# Autodesk Inventor assembly: UQ204-topHolder-sample
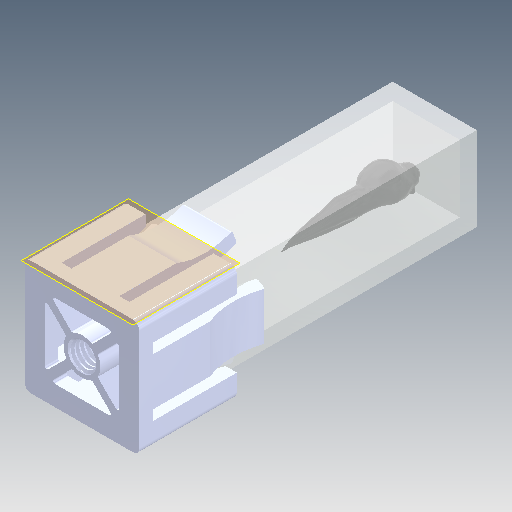
[picture p0: Inventor's stored thumbnail of the model, 512x512]
Saved by Autodesk Inventor 2021 (Build 250183000, 183)
## iProperties
Created: 2023-02-10
Part Number: UQ204-topHolder-sample
Document SubType Name: Assembly
Designer: nvladi
Author: nvladi
## Documents named in this file (4)
- C:\Users\Public\GitHub-public\benchtop-hardware\Benchtop\custom-parts\sample_handling\assemblies\UQ204-topHolder-sample.iam
- C:\Users\Public\GitHub-public\benchtop-hardware\Benchtop\CAD-model-Inventor2021\library\Portmann Instruments\UQ-204-10x10x45mm.ipt
- C:\Users\Public\GitHub-public\benchtop-hardware\Benchtop\custom-parts\sample_handling\cuvette-holders\Cuvette-12.5x12.5mm(UG204)\TopClamp-UG204_100943(Quadrat 2mm)_D.ipt
- C:\Users\Public\GitHub-public\benchtop-hardware\Benchtop\CAD-model-Inventor2021\library\samples\tadpole-20mm.ipt
## Components (3 placed, 3 different names)
1. UQ-204-10x10x45mm:1 — Mate:1
2. TopClamp-UG204_100943(Quadrat 2mm)_D:1 — Mate:1
3. tadpole-20mm:1
## Relationships (1: Mate 1)
- Mate:1: UQ-204-10x10x45mm:1 ↔ TopClamp-UG204_100943(Quadrat 2mm)_D:1
